# Autodesk Inventor assembly: EjeRueda
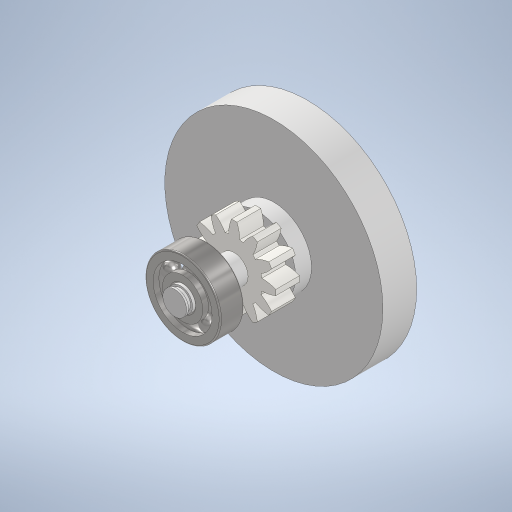
[picture p0: Inventor's stored thumbnail of the model, 512x512]
Saved by Autodesk Inventor 2023.1 (Build 271208000, 208)
## iProperties
Created: 2022-09-09
Part Number: EjeRueda
Document SubType Name: Assembly
Designer: Lab. de Manufactura
Author: Lab. de Manufactura
## Documents named in this file (5)
- C:\Users\Lab. de Manufactura\Desktop\SSL\Jean\EjeRueda.iam
- C:\Users\Lab. de Manufactura\Desktop\SSL\Jean\EjeSmallSize\eje.ipt
- C:\Users\Lab. de Manufactura\Desktop\SSL\Jean\omniwheel.ipt
- C:\Users\Lab. de Manufactura\Desktop\SSL\Jean\SmallSize\Design Accelerator\Engranaje recto11.ipt
- C:\Users\Lab. de Manufactura\Desktop\SSL\Jean\BS 290 SKF - SKF 626-2RS1.ipt
## Components (4 placed, 4 different names)
1. eje:1 — Rígido:1, Rígido:2, De rotación:1
2. omniwheel:1 — Rígido:1
3. Engranaje recto1:1 — Rígido:2
4. BS 290 SKF- con dos juntas RS1 SKF 626-2RS1:1 — De rotación:1
## Relationships (3: WeldJoint 2, RevoluteJoint 1)
- Rígido:1 [WeldJoint]: eje:1 ↔ omniwheel:1
- Rígido:2 [WeldJoint]: eje:1 ↔ Engranaje recto1:1
- De rotación:1 [RevoluteJoint]: eje:1 ↔ BS 290 SKF- con dos juntas RS1 SKF 626-2RS1:1
